# Autodesk Inventor assembly: 飛び出す奴
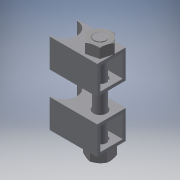
[picture p0: Inventor's stored thumbnail of the model, 180x180]
Saved by Autodesk Inventor 2018 (Build 220112000, 112)
## iProperties
Created: 2017-09-10
Part Number: 飛び出す奴
Material: 一般
Document SubType Name: Assembly
Designer: Kenta
Author: Kenta
## Documents named in this file (4)
- C:\Users\Kenta\Documents\workspace\rbbr\cart\シャーシ\飛び出す奴２.iam
- C:\Users\Kenta\Documents\workspace\rbbr\cart\シャーシ\左右に飛び出すパイプ.ipt
- C:\Users\Kenta\Documents\workspace\rbbr\cart\シャーシ\hn1_14.ipt
- C:\Users\Kenta\Documents\workspace\rbbr\cart\シャーシ\12mmパイプ.ipt
## Components (5 placed, 3 different names)
1. 左右に飛び出すパイプ:1 — フラッシュ:3, メイト:11
2. 左右に飛び出すパイプ:2 — フラッシュ:3, メイト:8
3. hn1_14:1 — メイト:7, メイト:9, フラッシュ:4
4. hn1_14:2 — メイト:10, フラッシュ:5
5. 12mmパイプ:1 — メイト:7, メイト:8, メイト:9, メイト:10, メイト:11, フラッシュ:4, フラッシュ:5
## Relationships (10: Mate 7, Flush 3)
- [Mate]: 左右に飛び出すパイプ:1 ↔ hn1_14:1
- [Mate]: 左右に飛び出すパイプ:2 ↔ hn1_14:2
- フラッシュ:3 [Flush]: 左右に飛び出すパイプ:1 ↔ 左右に飛び出すパイプ:2
- メイト:7 [Mate]: hn1_14:1 ↔ 12mmパイプ:1
- メイト:8 [Mate]: 左右に飛び出すパイプ:2 ↔ 12mmパイプ:1
- メイト:9 [Mate]: hn1_14:1 ↔ 12mmパイプ:1
- メイト:10 [Mate]: hn1_14:2 ↔ 12mmパイプ:1
- メイト:11 [Mate]: 左右に飛び出すパイプ:1 ↔ 12mmパイプ:1
- フラッシュ:4 [Flush]: hn1_14:1 ↔ 12mmパイプ:1
- フラッシュ:5 [Flush]: hn1_14:2 ↔ 12mmパイプ:1
